# Autodesk Inventor assembly: Geneva drive
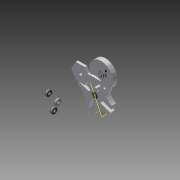
[picture p0: Inventor's stored thumbnail of the model, 180x180]
Saved by Autodesk Inventor 2018 (Build 220112000, 112)
## iProperties
Created: 2018-01-19
Part Number: Geneva drive
Document SubType Name: Assembly
Designer: Rus
Author: Rus
## Documents named in this file (6)
- E:\Libraries\3D Objects\Geneva drive\Mechanical\Attempt 2v2\Geneva drive Assembly.iam
- E:\Libraries\3D Objects\Geneva drive\Mechanical\Attempt 2v2\Geneva Drive.ipt
- E:\Libraries\3D Objects\Geneva drive\Mechanical\Attempt 2v2\Geneva Driven.ipt
- E:\Libraries\3D Objects\Geneva drive\Mechanical\Attempt 2v2\Frame.ipt
- E:\Libraries\3D Objects\Geneva drive\Mechanical\Attempt 2v2\608ZZ.iam
- E:\Libraries\3D Objects\Bearings\608\Driver Shaft.ipt
## Components (8 placed, 5 different names)
1. Geneva Drive:1 — Flush:1, Mate:1, Mate:2
2. Geneva Driven:1 — Insert:1
3. Frame:1
4. 608ZZ:1 [sub-assembly]
5. 608ZZ:2 [sub-assembly]
6. Driver Shaft:1 — Flush:1, Mate:1, Mate:2
7. 608ZZ:3 [sub-assembly]
8. 608ZZ:4 [sub-assembly] — Insert:1
## Relationships (4: Mate 2, Insert 1, Flush 1)
- Insert:1: Geneva Driven:1 ↔ 608ZZ:4
- Flush:1: Geneva Drive:1 ↔ Driver Shaft:1
- Mate:1: Geneva Drive:1 ↔ Driver Shaft:1
- Mate:2: Geneva Drive:1 ↔ Driver Shaft:1
